# Autodesk Inventor assembly: V3Intake
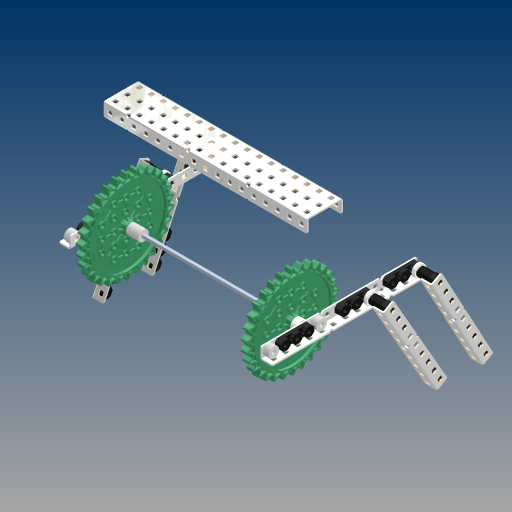
[picture p0: Inventor's stored thumbnail of the model, 512x512]
Saved by Autodesk Inventor 2023 (Build 270158000, 158)
## iProperties
Created: 2023-08-05
Part Number: V3Intake
Document SubType Name: Assembly
Designer: eddie
Author: eddie
## Documents named in this file (17)
- C:\Users\eddie\Documents\81208X-Over-Under-CAD\V3\V3Intake.iam
- C:\Users\eddie\Documents\81208X-Over-Under-CAD\VEX-CAD-Inventor-1.4.0\Structure\Angle\Aluminum\1x1\Alu Angle 1x1x13.ipt
- C:\Users\eddie\Documents\81208X-Over-Under-CAD\VEX-CAD-Inventor-1.4.0\Structure\C Channel\Aluminum 1x3x1\Alu C 1x3x1x17.ipt
- C:\Users\eddie\Documents\81208X-Over-Under-CAD\VEX-CAD-Inventor-1.4.0\Motion\Shaft LS\Bearing Flat.ipt
- C:\Users\eddie\Documents\81208X-Over-Under-CAD\Custom-parts\Shaft Collar.ipt
- C:\Users\eddie\Documents\81208X-Over-Under-CAD\VEX-CAD-Inventor-1.4.0\Motion\Shaft LS\Shaft LS\Shaft LS 8.0.ipt
- C:\Users\eddie\Documents\81208X-Over-Under-CAD\VEX-CAD-Inventor-1.4.0\Motion\Shaft LS\Shaft LS.ipt
- C:\Users\eddie\Documents\81208X-Over-Under-CAD\VEX-CAD-Inventor-1.4.0\Motion\Spacers\Spacer Nylon .500 OD\NSpacer White .500 OD x .250.ipt
- C:\Users\eddie\Documents\81208X-Over-Under-CAD\VEX-CAD-Inventor-1.4.0\Motion\Spacers\Spacer Nylon .500 OD.ipt
- C:\Users\eddie\Documents\81208X-Over-Under-CAD\VEX-CAD-Inventor-1.4.0\Motion\Sprockets\9P Sprocket\9P 30T Sprocket, Square.iam
- C:\Users\eddie\Documents\81208X-Over-Under-CAD\VEX-CAD-Inventor-1.4.0\Motion\Sprockets\9P Sprocket.iam
- C:\Users\eddie\Documents\81208X-Over-Under-CAD\VEX-CAD-Inventor-1.4.0\Structure\Angle\Aluminum\1x1\Alu Angle 1x1x9.ipt
- C:\Users\eddie\Documents\81208X-Over-Under-CAD\VEX-CAD-Inventor-1.4.0\Motion\Spacers\Spacer Nylon .500 OD\NSpacer White .500 OD x .125.ipt
- C:\Users\eddie\Documents\81208X-Over-Under-CAD\VEX-CAD-Inventor-1.4.0\Motion\Spacers\Washer Steel\SWasher .375 OD x .031250.ipt
- C:\Users\eddie\Documents\81208X-Over-Under-CAD\VEX-CAD-Inventor-1.4.0\Motion\Spacers\Washer Steel.ipt
- C:\Users\eddie\Documents\81208X-Over-Under-CAD\VEX-CAD-Inventor-1.4.0\Motion\Spacers\Spacer Nylon .375 OD\NSpacer .375 OD x .500.ipt
- C:\Users\eddie\Documents\81208X-Over-Under-CAD\VEX-CAD-Inventor-1.4.0\Motion\Spacers\Spacer Nylon .375 OD.ipt
## Components (46 placed, 11 different names)
1. Alu Angle 1x1x13:1 — Insert:1, Insert:2, Insert:3, Insert:7, Insert:8, Insert:14
2. Alu Angle 1x1x13:2 — Insert:4, Insert:5, Insert:6, Insert:9, Insert:10, Insert:12, Insert:13
3. Alu C 1x3x1x17:1
4. Bearing Flat:1 — Insert:1, Insert:31
5. Bearing Flat:2 — Insert:2, Insert:21
6. Bearing Flat:3 — Insert:3, Insert:11
7. Bearing Flat:4 — Insert:4, Insert:37
8. Bearing Flat:5 — Insert:5, Insert:38
9. Bearing Flat:6 — Insert:6
10. Shaft Collar:1 — Insert:7
11. Shaft Collar:2 — Insert:8
12. Shaft Collar:3 — Insert:9
13. Shaft Collar:4 — Insert:10
14. Shaft LS 8.0:1 — Insert:11, Insert:12
15. NSpacer White .500 OD x .250:1 — Insert:13, Insert:16
16. NSpacer White .500 OD x .250:2 — Insert:14, Insert:15
17. 9P 30T Sprocket, Square:1 [sub-assembly] — Insert:15, Insert:19
18. 9P 30T Sprocket, Square:2 [sub-assembly] — Insert:16, Insert:17
19. Shaft Collar:5 — Insert:18
20. Shaft Collar:6 — Insert:17, Insert:18
21. Shaft Collar:7 — Insert:19, Insert:20
22. Shaft Collar:8 — Insert:20
23. Alu Angle 1x1x9:1 — Insert:24, Insert:25, Insert:29, Insert:30
24. Alu Angle 1x1x9:2 — Insert:26, Insert:27, Insert:35, Insert:36
25. NSpacer White .500 OD x .125:3 — Insert:21, Insert:22
26. SWasher .375 OD x .031250:1 — Insert:22, Insert:23
27. NSpacer .375 OD x .500:1 — Insert:23, Insert:28
28. Bearing Flat:7 — Insert:24, Insert:28, Insert:29
29. Bearing Flat:8 — Insert:25, Insert:30
30. Bearing Flat:9 — Insert:26, Insert:34, Insert:35
31. Bearing Flat:10 — Insert:27, Insert:36
32. NSpacer White .500 OD x .125:4 — Insert:31, Insert:32
33. SWasher .375 OD x .031250:2 — Insert:32, Insert:33
34. NSpacer .375 OD x .500:2 — Insert:33, Insert:34
35. Alu Angle 1x1x9:4 — Insert:45, Insert:46, Insert:49, Insert:50
36. Alu Angle 1x1x9:5 — Insert:43, Insert:44, Insert:47, Insert:48
37. NSpacer White .500 OD x .125:5 — Insert:37, Insert:39
38. NSpacer White .500 OD x .125:6 — Insert:38, Insert:40
39. SWasher .375 OD x .031250:3 — Insert:39, Insert:42
40. SWasher .375 OD x .031250:4 — Insert:40, Insert:41
41. NSpacer .375 OD x .500:3 — Insert:42, Insert:52
42. NSpacer .375 OD x .500:4 — Insert:41, Insert:51
43. Bearing Flat:11 — Insert:43, Insert:47, Insert:52
44. Bearing Flat:12 — Insert:44, Insert:48
45. Bearing Flat:13 — Insert:46, Insert:50
46. Bearing Flat:14 — Insert:45, Insert:49, Insert:51
## Relationships (52: Insert 52)
- Insert:1: Alu Angle 1x1x13:1 ↔ Bearing Flat:1
- Insert:2: Alu Angle 1x1x13:1 ↔ Bearing Flat:2
- Insert:3: Alu Angle 1x1x13:1 ↔ Bearing Flat:3
- Insert:4: Alu Angle 1x1x13:2 ↔ Bearing Flat:4
- Insert:5: Alu Angle 1x1x13:2 ↔ Bearing Flat:5
- Insert:6: Alu Angle 1x1x13:2 ↔ Bearing Flat:6
- Insert:7: Alu Angle 1x1x13:1 ↔ Shaft Collar:1
- Insert:8: Alu Angle 1x1x13:1 ↔ Shaft Collar:2
- Insert:9: Alu Angle 1x1x13:2 ↔ Shaft Collar:3
- Insert:10: Alu Angle 1x1x13:2 ↔ Shaft Collar:4
- Insert:11: Bearing Flat:3 ↔ Shaft LS 8.0:1
- Insert:12: Alu Angle 1x1x13:2 ↔ Shaft LS 8.0:1
- Insert:13: Alu Angle 1x1x13:2 ↔ NSpacer White .500 OD x .250:1
- Insert:14: Alu Angle 1x1x13:1 ↔ NSpacer White .500 OD x .250:2
- Insert:15: NSpacer White .500 OD x .250:2 ↔ 9P 30T Sprocket, Square:1
- Insert:16: NSpacer White .500 OD x .250:1 ↔ 9P 30T Sprocket, Square:2
- Insert:17: 9P 30T Sprocket, Square:2 ↔ Shaft Collar:6
- Insert:18: Shaft Collar:5 ↔ Shaft Collar:6
- Insert:19: 9P 30T Sprocket, Square:1 ↔ Shaft Collar:7
- Insert:20: Shaft Collar:7 ↔ Shaft Collar:8
- Insert:21: Bearing Flat:2 ↔ NSpacer White .500 OD x .125:3
- Insert:22: NSpacer White .500 OD x .125:3 ↔ SWasher .375 OD x .031250:1
- Insert:23: SWasher .375 OD x .031250:1 ↔ NSpacer .375 OD x .500:1
- Insert:24: Alu Angle 1x1x9:1 ↔ Bearing Flat:7
- Insert:25: Alu Angle 1x1x9:1 ↔ Bearing Flat:8
- Insert:26: Alu Angle 1x1x9:2 ↔ Bearing Flat:9
- Insert:27: Alu Angle 1x1x9:2 ↔ Bearing Flat:10
- Insert:28: NSpacer .375 OD x .500:1 ↔ Bearing Flat:7
- Insert:29: Alu Angle 1x1x9:1 ↔ Bearing Flat:7
- Insert:30: Alu Angle 1x1x9:1 ↔ Bearing Flat:8
- Insert:31: Bearing Flat:1 ↔ NSpacer White .500 OD x .125:4
- Insert:32: NSpacer White .500 OD x .125:4 ↔ SWasher .375 OD x .031250:2
- Insert:33: SWasher .375 OD x .031250:2 ↔ NSpacer .375 OD x .500:2
- Insert:34: Bearing Flat:9 ↔ NSpacer .375 OD x .500:2
- Insert:35: Alu Angle 1x1x9:2 ↔ Bearing Flat:9
- Insert:36: Alu Angle 1x1x9:2 ↔ Bearing Flat:10
- Insert:37: Bearing Flat:4 ↔ NSpacer White .500 OD x .125:5
- Insert:38: Bearing Flat:5 ↔ NSpacer White .500 OD x .125:6
- Insert:39: NSpacer White .500 OD x .125:5 ↔ SWasher .375 OD x .031250:3
- Insert:40: NSpacer White .500 OD x .125:6 ↔ SWasher .375 OD x .031250:4
- Insert:41: SWasher .375 OD x .031250:4 ↔ NSpacer .375 OD x .500:4
- Insert:42: SWasher .375 OD x .031250:3 ↔ NSpacer .375 OD x .500:3
- Insert:43: Alu Angle 1x1x9:5 ↔ Bearing Flat:11
- Insert:44: Alu Angle 1x1x9:5 ↔ Bearing Flat:12
- Insert:45: Alu Angle 1x1x9:4 ↔ Bearing Flat:14
- Insert:46: Alu Angle 1x1x9:4 ↔ Bearing Flat:13
- Insert:47: Alu Angle 1x1x9:5 ↔ Bearing Flat:11
- Insert:48: Alu Angle 1x1x9:5 ↔ Bearing Flat:12
- Insert:49: Alu Angle 1x1x9:4 ↔ Bearing Flat:14
- Insert:50: Alu Angle 1x1x9:4 ↔ Bearing Flat:13
- Insert:51: NSpacer .375 OD x .500:4 ↔ Bearing Flat:14
- Insert:52: NSpacer .375 OD x .500:3 ↔ Bearing Flat:11
